# Autodesk Inventor assembly: TopPlate
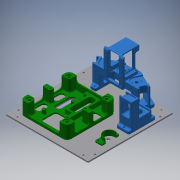
[picture p0: Inventor's stored thumbnail of the model, 180x180]
Saved by Autodesk Inventor 2016 (Build 200138000, 138)
## iProperties
Created: 2015-08-28
Part Number: TopPlate
Document SubType Name: Assembly
Designer: lachesis
Author: lachesis
## Documents named in this file (7)
- C:\Users\lachesis\git\Swarmie-Build\Swarmie-Assembly\Assemblies\TopPlate.iam
- C:\Users\lachesis\git\Swarmie-Build\Swarmie-Assembly\Parts\TopPlate.ipt
- C:\Users\lachesis\git\Swarmie-Build\Swarmie-Assembly\Parts\USTowerLW.ipt
- C:\Users\lachesis\git\Swarmie-Build\Swarmie-Assembly\Parts\CameraMountLW.ipt
- C:\Users\lachesis\git\Swarmie-Build\Swarmie-Assembly\Parts\SwitchGuardLW.ipt
- C:\Users\lachesis\git\Swarmie-Build\Swarmie-Assembly\Parts\GPS_IMUMountLW.ipt
- C:\Users\lachesis\git\Swarmie-Build\Swarmie-Assembly\Parts\NUCBaseLW.ipt
## Components (6 placed, 6 different names)
1. TopPlate:1 — Rigid:2, Rigid:3, Rigid:4, Rigid:5
2. GPS_IMUMountLW:1 — Rigid:2
3. NUCBaseLW:1 — Rigid:3
4. SwitchGuardLW:1 — Rigid:4
5. USTowerLW:1 — Rigid:5, Rigid:6
6. CameraMountLW:1 — Rigid:6
## Relationships (5: WeldJoint 5)
- Rigid:2 [WeldJoint]: TopPlate:1 ↔ GPS_IMUMountLW:1
- Rigid:3 [WeldJoint]: TopPlate:1 ↔ NUCBaseLW:1
- Rigid:4 [WeldJoint]: TopPlate:1 ↔ SwitchGuardLW:1
- Rigid:5 [WeldJoint]: TopPlate:1 ↔ USTowerLW:1
- Rigid:6 [WeldJoint]: USTowerLW:1 ↔ CameraMountLW:1
